# Autodesk Inventor assembly: leg_1_MIR
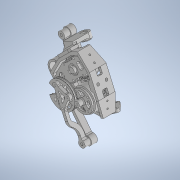
[picture p0: Inventor's stored thumbnail of the model, 180x180]
Saved by Autodesk Inventor 2020 (Build 240168000, 168)
## iProperties
Created: 2020-12-08
Part Number: leg_1_MIR
Document SubType Name: Assembly
Designer: Shuang Peng
Author: Shuang Peng
## Documents named in this file (11)
- D:\projects-3\biped_tiny\hardware\sim_mod\leg_1_MIR_sim.iam
- D:\projects-3\biped_tiny\hardware\leg_holder_2_MIR.ipt
- D:\projects-3\biped_tiny\hardware\leg_link_1_MIR.ipt
- D:\projects-3\biped_tiny\hardware\leg_link_2_MIR.ipt
- D:\projects-3\biped_tiny\hardware\leg_link_4_MIR.ipt
- D:\projects-3\biped_tiny\hardware\leg_link_3_m_MIR.ipt
- D:\projects-3\biped_tiny\hardware\foot_2_MIR.ipt
- D:\projects-3\biped_tiny\hardware\pin_3_15_MIR.ipt
- D:\projects-3\biped_tiny\hardware\body_conn_1_MIR.ipt
- D:\projects-3\biped_tiny\hardware\sim_mod\reducer_1.iam
- D:\projects-3\biped_tiny\hardware\body_conn_2_MIR.ipt
## Components (14 placed, 10 different names)
1. leg_holder_2_MIR:1 — Insert:28, Insert:29, Insert:30, Insert:31, Insert:32, Insert:33, Insert:37, Insert:38, Angle:1, Angle:2
2. leg_link_1_MIR:1 — Flush:5, Insert:9, Flush:6, Insert:16, Insert:19, Insert:18, Flush:7
3. leg_link_2_MIR:1 — Insert:9, Flush:6, Insert:26, Insert:35, Angle:1
4. leg_link_4_MIR:1 — Insert:17, Insert:34, Angle:2
5. leg_link_3_m_MIR:1 — Insert:17, Insert:16, Insert:27, Insert:28
6. foot_2_MIR:1 — Insert:19, Insert:18, Flush:7
7. pin_3_15_MIR:1 — Insert:26
8. pin_3_15_MIR:2 — Insert:27
9. pin_3_15_MIR:3 — Insert:28
10. body_conn_1_MIR:1 — Insert:28, Insert:29, Insert:36
11. reducer_1:1 [sub-assembly] — Insert:32, Insert:33, Insert:34
12. reducer_1:2 [sub-assembly] — Insert:30, Insert:31, Insert:35
13. pin_3_15_MIR:4 — Insert:36
14. body_conn_2_MIR:1 — Insert:37, Insert:38
## Relationships (24: Insert 19, Mate 3, Angle 2)
- Flush:5 [Mate]: leg_link_1_MIR:1
- Insert:9: leg_link_1_MIR:1 ↔ leg_link_2_MIR:1
- Flush:6 [Mate]: leg_link_1_MIR:1 ↔ leg_link_2_MIR:1
- Insert:17: leg_link_4_MIR:1 ↔ leg_link_3_m_MIR:1
- Insert:16: leg_link_1_MIR:1 ↔ leg_link_3_m_MIR:1
- Insert:19: leg_link_1_MIR:1 ↔ foot_2_MIR:1
- Insert:18: leg_link_1_MIR:1 ↔ foot_2_MIR:1
- Flush:7 [Mate]: leg_link_1_MIR:1 ↔ foot_2_MIR:1
- Insert:26: leg_link_2_MIR:1 ↔ pin_3_15_MIR:1
- Insert:27: leg_link_3_m_MIR:1 ↔ pin_3_15_MIR:2
- Insert:28: leg_link_3_m_MIR:1 ↔ pin_3_15_MIR:3
- Insert:28: leg_holder_2_MIR:1 ↔ body_conn_1_MIR:1
- Insert:29: leg_holder_2_MIR:1 ↔ body_conn_1_MIR:1
- Insert:30: leg_holder_2_MIR:1 ↔ reducer_1:2
- Insert:31: leg_holder_2_MIR:1 ↔ reducer_1:2
- Insert:32: leg_holder_2_MIR:1 ↔ reducer_1:1
- Insert:33: leg_holder_2_MIR:1 ↔ reducer_1:1
- Insert:34: leg_link_4_MIR:1 ↔ reducer_1:1
- Insert:35: leg_link_2_MIR:1 ↔ reducer_1:2
- Insert:36 (-12 mm): body_conn_1_MIR:1 ↔ pin_3_15_MIR:4
- Insert:37: leg_holder_2_MIR:1 ↔ body_conn_2_MIR:1
- Insert:38: leg_holder_2_MIR:1 ↔ body_conn_2_MIR:1
- Angle:1 (0 deg): leg_holder_2_MIR:1 ↔ leg_link_2_MIR:1
- Angle:2 (0 deg): leg_holder_2_MIR:1 ↔ leg_link_4_MIR:1
